# Autodesk Inventor assembly: splashAssembly
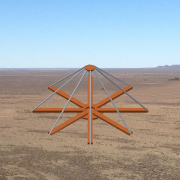
[picture p0: Inventor's stored thumbnail of the model, 180x180]
Saved by Autodesk Inventor 2014 SP1 (Build 180222100, 222)
## iProperties
Created: 2013-06-11
Part Number: splashAssembly
Document SubType Name: Assembly
Designer: Dave
Author: Dave
## Documents named in this file (6)
- C:\Users\Dave\Desktop\hera-cad\surface\splashAssembly.iam
- C:\Users\Dave\Desktop\hera-cad\surface\splash_base.ipt
- C:\Users\Dave\Desktop\hera-cad\surface\splash_shortPVC.ipt
- C:\Users\Dave\Desktop\hera-cad\surface\splash_top.ipt
- C:\Users\Dave\Desktop\hera-cad\surface\splashBase.iam
- C:\Users\Dave\Desktop\hera-cad\surface\splashTopDisc.ipt
## Components (12 placed, 5 different names)
1. splash_base:1 — Insert:1
2. splash_top:1 — Insert:1
3. splashBase:1 [sub-assembly]
4. splashTopDisc:1
5. splash_shortPVC:1
6. splash_shortPVC:2
7. splash_shortPVC:3
8. splash_shortPVC:4
9. splash_shortPVC:5
10. splash_shortPVC:6
11. splash_shortPVC:7
12. splash_shortPVC:8
## Component patterns: (8 elements, first: splash_shortPVC:1)
## Relationships (1: Insert 1)
- Insert:1 (12.7 mm): splash_base:1 ↔ splash_top:1
